# Autodesk Inventor assembly: HACKberry_R
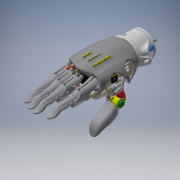
[picture p0: Inventor's stored thumbnail of the model, 180x180]
Saved by Autodesk Inventor 2018.1 (Build 221171000, 171)
## iProperties
Created: 2017-09-19
Part Number: HACKberry_R
Material: 一般
Document SubType Name: Assembly
Designer: sktom
Sending System: Autodesk Translation Framework v6.1.1.50
Preprocessor: ST-DEVELOPER v16.13
Title: c:\worker\convert-fusion-sep-2017\tmp\job-1\7\output\files\eae90a9c-ec5b-42e5-911f-74c536a00ecb\690ac6e2-c184-4c90-b615-a54286bbc40c.stp
## Documents named in this file (3)
- D:\CloudStrage\NextCloud\Cad_mechanical\HACKberry_SizeM\3Dmodel\R\HACKberry_R.iam
- D:\CloudStrage\NextCloud\Cad_mechanical\HACKberry_SizeM\3Dmodel\R\M-R-H\M-R-H.iam
- D:\CloudStrage\NextCloud\Cad_mechanical\HACKberry_SizeM\3Dmodel\R\M-R-W\M-R-W.iam
## Components (2 placed, 2 different names)
1. M-R-H:1 [sub-assembly] — 挿入:1
2. M-R-W:1 [sub-assembly] — 挿入:1
## Relationships (1: Insert 1)
- 挿入:1 [Insert]: M-R-H:1 ↔ M-R-W:1
